# Autodesk Inventor assembly: Tool Rack Assembly
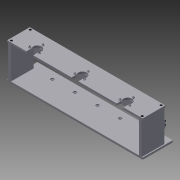
[picture p0: Inventor's stored thumbnail of the model, 180x180]
Saved by Autodesk Inventor 2012 SP1 (Build 160190100, 190)
## iProperties
Created: 2010-12-14
Part Number: Tool Rack Assembly
Document SubType Name: Assembly
Designer: berny
Author: berny
## Documents named in this file (9)
- D:\Users\ding42\Dropbox\Inventor files\CMS\Module Assembly Station\Gantry\NewGantryParts\Gantry Full Assembly\Tool Rack\Tool Rack Assembly.iam
- D:\Users\ding42\Dropbox\Inventor files\CMS\Module Assembly Station\Gantry\NewGantryParts\Gantry Full Assembly\Tool Rack\Bottom.ipt
- D:\Users\ding42\Dropbox\Inventor files\CMS\Module Assembly Station\Gantry\NewGantryParts\Gantry Full Assembly\Tool Rack\Sides.ipt
- D:\Users\ding42\Dropbox\Inventor files\CMS\Module Assembly Station\Gantry\NewGantryParts\Gantry Full Assembly\Tool Rack\Top.ipt
- D:\Users\ding42\Dropbox\Inventor files\CMS\Module Assembly Station\Gantry\NewGantryParts\Gantry Full Assembly\Tool Rack\BackStrap1.ipt
- D:\Users\ding42\Dropbox\Inventor files\CMS\Module Assembly Station\Gantry\NewGantryParts\NewParts\SHCS-steel 8-32x0.5.ipt
- D:\Inventor\iParts\Fasteners\Bolt-SHCS.ipt
- D:\Users\ding42\Dropbox\Inventor files\CMS\Module Assembly Station\Gantry\NewGantryParts\Gantry Full Assembly\Tool Rack\84985A58.iam
- D:\Users\ding42\Dropbox\Inventor files\CMS\Module Assembly Station\Gantry\NewGantryParts\Gantry Full Assembly\Tool Rack\84985A15.iam
## Components (26 placed, 7 different names)
1. Top:1 — Mate:3, Flush:13, Flush:14, Flush:15, Flush:16, Insert:21, Insert:22, Insert:23, Insert:24, Insert:33, Insert:34, Insert:35, Insert:36, Insert:37, Insert:38, Insert:39, Insert:41, Insert:42
2. Sides:1 — Mate:2, Flush:3, Flush:4, Mate:3, Flush:13, Flush:14, Mate:14
3. Sides:2 — Mate:1, Flush:15, Flush:16, Flush:17, Mate:15
4. Bottom:1 — Mate:1, Mate:2, Flush:3, Flush:4, Insert:25, Insert:26, Insert:27, Insert:28
5. BackStrap1:1 — Mate:14, Flush:17, Mate:15, Insert:29, Insert:30, Insert:31, Insert:32
6. SHCS-steel 8-32x0.5:1 — Insert:21
7. SHCS-steel 8-32x0.5:2 — Insert:22
8. SHCS-steel 8-32x0.5:3 — Insert:28
9. SHCS-steel 8-32x0.5:4 — Insert:32
10. SHCS-steel 8-32x0.5:5 — Insert:25
11. SHCS-steel 8-32x0.5:6 — Insert:31
12. SHCS-steel 8-32x0.5:7 — Insert:30
13. SHCS-steel 8-32x0.5:8 — Insert:29
14. SHCS-steel 8-32x0.5:9 — Insert:27
15. SHCS-steel 8-32x0.5:10 — Insert:26
16. SHCS-steel 8-32x0.5:11 — Insert:24
17. SHCS-steel 8-32x0.5:12 — Insert:23
18. 84985A58:1 [sub-assembly] — Insert:36
19. 84985A58:2 [sub-assembly] — Insert:38
20. 84985A58:3 [sub-assembly] — Insert:37
21. 84985A58:4 [sub-assembly] — Insert:42
22. 84985A58:5 [sub-assembly] — Insert:41
23. 84985A58:6 [sub-assembly] — Insert:39
24. 84985A15:1 [sub-assembly] — Insert:33
25. 84985A15:2 [sub-assembly] — Insert:34
26. 84985A15:3 [sub-assembly] — Insert:35
## Relationships (33: Insert 21, Flush 7, Mate 5)
- Mate:1: Sides:2 ↔ Bottom:1
- Mate:2: Sides:1 ↔ Bottom:1
- Flush:3: Sides:1 ↔ Bottom:1
- Flush:4 (3.175 mm): Sides:1 ↔ Bottom:1
- Mate:3: Top:1 ↔ Sides:1
- Flush:13 (-3.175 mm): Top:1 ↔ Sides:1
- Flush:14: Top:1 ↔ Sides:1
- Flush:15 (3.175 mm): Top:1 ↔ Sides:2
- Flush:16: Top:1 ↔ Sides:2
- Mate:14: Sides:1 ↔ BackStrap1:1
- Flush:17: Sides:2 ↔ BackStrap1:1
- Mate:15: Sides:2 ↔ BackStrap1:1
- Insert:21: Top:1 ↔ SHCS-steel 8-32x0.5:1
- Insert:22: Top:1 ↔ SHCS-steel 8-32x0.5:2
- Insert:23: Top:1 ↔ SHCS-steel 8-32x0.5:12
- Insert:24: Top:1 ↔ SHCS-steel 8-32x0.5:11
- Insert:25: Bottom:1 ↔ SHCS-steel 8-32x0.5:5
- Insert:26: Bottom:1 ↔ SHCS-steel 8-32x0.5:10
- Insert:27: Bottom:1 ↔ SHCS-steel 8-32x0.5:9
- Insert:28: Bottom:1 ↔ SHCS-steel 8-32x0.5:3
- Insert:29: BackStrap1:1 ↔ SHCS-steel 8-32x0.5:8
- Insert:30: BackStrap1:1 ↔ SHCS-steel 8-32x0.5:7
- Insert:31: BackStrap1:1 ↔ SHCS-steel 8-32x0.5:6
- Insert:32: BackStrap1:1 ↔ SHCS-steel 8-32x0.5:4
- Insert:33 (-5.08 mm): Top:1 ↔ 84985A15:1
- Insert:34 (-5.08 mm): Top:1 ↔ 84985A15:2
- Insert:35 (-5.08 mm): Top:1 ↔ 84985A15:3
- Insert:36 (-5.08 mm): Top:1 ↔ 84985A58:1
- Insert:37 (-5.08 mm): Top:1 ↔ 84985A58:3
- Insert:38 (-5.08 mm): Top:1 ↔ 84985A58:2
- Insert:39 (-5.08 mm): Top:1 ↔ 84985A58:6
- Insert:41 (-5.08 mm): Top:1 ↔ 84985A58:5
- Insert:42 (-5.08 mm): Top:1 ↔ 84985A58:4
